# Autodesk Inventor assembly: Assembly4
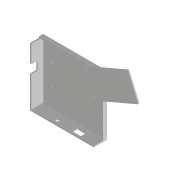
[picture p0: Inventor's stored thumbnail of the model, 180x180]
Saved by Autodesk Inventor 2020 (Build 240168000, 168)
## iProperties
Created: 2020-11-12
Part Number: Assembly4
Document SubType Name: Assembly
Designer: ferrerx
Author: ferrerx
## Documents named in this file (7)
- C:\Users\ferrerx\Desktop\Projects\Prieto-Godino Lab\Drosophila Larvae Behavioural Device\Device design V3\Electronics case\Assembly4.iam
- C:\Users\ferrerx\Desktop\Projects\Prieto-Godino Lab\Drosophila Larvae Behavioural Device\Device design V3\Electronics case\Base.ipt
- C:\Users\ferrerx\Desktop\Projects\Prieto-Godino Lab\Drosophila Larvae Behavioural Device\Device design V3\Electronics case\Lateral Power supply.ipt
- C:\Users\ferrerx\Desktop\Projects\Prieto-Godino Lab\Drosophila Larvae Behavioural Device\Device design V3\Electronics case\Spacer.ipt
- C:\Users\ferrerx\Desktop\Projects\Prieto-Godino Lab\Drosophila Larvae Behavioural Device\Device design V3\Electronics case\Lateral USB.ipt
- C:\Users\ferrerx\Desktop\Projects\Prieto-Godino Lab\Drosophila Larvae Behavioural Device\Device design V3\Electronics case\Lateral Potentiometers.ipt
- C:\Users\ferrerx\Desktop\Projects\Prieto-Godino Lab\Drosophila Larvae Behavioural Device\Device design V3\Electronics case\Lateral Potentiometers short.ipt
## Components (6 placed, 6 different names)
1. Base:1 — Mate:6, Mate:7, Mate:8, Mate:15, Mate:16, Mate:20, Mate:21, Mate:22, Mate:23, Mate:24, Mate:25, Mate:26, Mate:27
2. Lateral Power supply:1 — Mate:6, Mate:7, Mate:8
3. Spacer:2 — Mate:15, Mate:16
4. Lateral USB:1 — Mate:20, Mate:21, Mate:22, Flush:1
5. Lateral Potentiometers:2 — Mate:23, Mate:24, Flush:1
6. Lateral Potentiometers short:1 — Mate:25, Mate:26, Mate:27
## Relationships (14: Mate 13, Flush 1)
- Mate:6: Base:1 ↔ Lateral Power supply:1
- Mate:7: Base:1 ↔ Lateral Power supply:1
- Mate:8: Base:1 ↔ Lateral Power supply:1
- Mate:15: Base:1 ↔ Spacer:2
- Mate:16: Base:1 ↔ Spacer:2
- Mate:20: Base:1 ↔ Lateral USB:1
- Mate:21: Base:1 ↔ Lateral USB:1
- Mate:22: Base:1 ↔ Lateral USB:1
- Mate:23: Base:1 ↔ Lateral Potentiometers:2
- Mate:24: Base:1 ↔ Lateral Potentiometers:2
- Flush:1: Lateral USB:1 ↔ Lateral Potentiometers:2
- Mate:25: Base:1 ↔ Lateral Potentiometers short:1
- Mate:26: Base:1 ↔ Lateral Potentiometers short:1
- Mate:27: Base:1 ↔ Lateral Potentiometers short:1
